# Autodesk Inventor assembly: model_awds
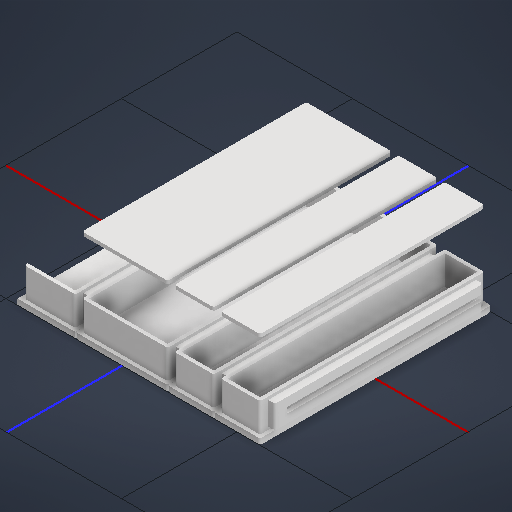
[picture p0: Inventor's stored thumbnail of the model, 512x512]
Saved by Autodesk Inventor 2025.2 (Build 292293000, 293)
## iProperties
Created: 2025-09-05
Part Number: model_awds
Document SubType Name: Assembly
Designer: sam
Author: sam
## Documents named in this file (6)
- G:\projects\primary\auto-water-distribution-system\model\asm\model_awds.iam
- G:\projects\primary\auto-water-distribution-system\model\asm\modules\module_command.ipt
- G:\projects\primary\auto-water-distribution-system\model\asm\modules\module-lid_command.ipt
- G:\projects\primary\auto-water-distribution-system\model\asm\modules\module_switch.ipt
- G:\projects\primary\auto-water-distribution-system\model\asm\modules\module-lid_switch.ipt
- G:\projects\primary\auto-water-distribution-system\model\asm\modules\module_valve.ipt
## Components (7 placed, 5 different names)
1. module_command:1 — Mate:1, Mate:2, Flush:1, Flush:2, Mate:11, Mate:12, Flush:5, Mate:15, Mate:16
2. module-lid_command:1 — Mate:1, Mate:2, Flush:3, Flush:4
3. module_switch:1 — Flush:1, Mate:7, Mate:8, Mate:11, Mate:12, Mate:13, Mate:14
4. module_switch:2 — Flush:2, Mate:9, Mate:10, Mate:13, Mate:14
5. module-lid_switch:1 — Flush:3, Mate:7, Mate:8
6. module-lid_switch:2 — Flush:4, Mate:9, Mate:10
7. module_valve:1 — Flush:5, Mate:15, Mate:16
## Relationships (17: Mate 12, Flush 5)
- Mate:1: module_command:1 ↔ module-lid_command:1
- Mate:2: module_command:1 ↔ module-lid_command:1
- Flush:1: module_command:1 ↔ module_switch:1
- Flush:2: module_command:1 ↔ module_switch:2
- Flush:3: module-lid_command:1 ↔ module-lid_switch:1
- Flush:4: module-lid_command:1 ↔ module-lid_switch:2
- Mate:7: module_switch:1 ↔ module-lid_switch:1
- Mate:8: module_switch:1 ↔ module-lid_switch:1
- Mate:9: module_switch:2 ↔ module-lid_switch:2
- Mate:10: module_switch:2 ↔ module-lid_switch:2
- Mate:11: module_command:1 ↔ module_switch:1
- Mate:12: module_command:1 ↔ module_switch:1
- Mate:13: module_switch:1 ↔ module_switch:2
- Mate:14: module_switch:1 ↔ module_switch:2
- Flush:5: module_command:1 ↔ module_valve:1
- Mate:15: module_command:1 ↔ module_valve:1
- Mate:16: module_command:1 ↔ module_valve:1
